# Autodesk Inventor assembly: Chassis-ver10-1111-2019
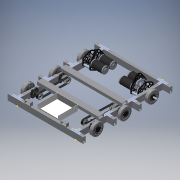
[picture p0: Inventor's stored thumbnail of the model, 180x180]
Saved by Autodesk Inventor 2018 (Build 220112000, 112)
## iProperties
Created: 2019-10-10
Part Number: Chassis-ver10-1111-2019
Document SubType Name: Assembly
Designer: JMHal
Author: JMHal
## Documents named in this file (30)
- F:\GrabCad\2019 - 2020 Off Season\TestChassis\Assembly\Chassis-ver10-1111-2019.iam
- F:\GrabCad\2019 - 2020 Off Season\TestChassis\Parts\2x1 20in Alluminum with Cal Drop.ver1-1111-2019.ipt
- F:\GrabCad\2019 - 2020 Off Season\TestChassis\Parts\2x1 20in Alluminum.ver1-1111-2019.ipt
- F:\GrabCad\2019 - 2020 Off Season\TestChassis\Parts\2x1 2in Alluminum Block.ver1-1111-2019.ipt
- F:\GrabCad\Resources\VEXpro Resources\Bearings\0.5inHexFlangedBearing(1.125inx0.313in)-1111-2016.ipt
- F:\GrabCad\Resources\VEXpro Resources\Versa Motion\VersaBlockKit-1111-2016.ipt
- F:\GrabCad\Resources\VEXpro Resources\Wheels\4 inch\4x1inTractionWheel(Tire)-1111-2016.iam
- F:\GrabCad\Resources\VEXpro Resources\Shafts\0.5inThunderHexShaft(8)-1111-2016.ipt
- F:\GrabCad\Resources\VEXpro Resources\Gearboxes\WCP SS Gearbox\SS-Gearbox.iam
- F:\GrabCad\Resources\VEXpro Resources\Gussets\ChassisGusset-1111-2016.ipt
- F:\GrabCad\2019 - 2020 Off Season\TestChassis\Parts\ElectricalBoardSupport.ver1-1111-2019.ipt
- F:\GrabCad\2019 - 2020 Off Season\TestChassis\Parts\ElectricalBoard.ver1-1111-2019.ipt
- F:\GrabCad\Resources\VEXpro Resources\Spacers\0.5inAcetalSpace(0.5inHex)-1111-2016.ipt
- F:\GrabCad\Resources\VEXpro Resources\Shafts\0.5inThunderHexShaft(8)-1111-2016_MIR.ipt
- F:\GrabCad\Resources\VEXpro Resources\Wheels\4 inch\4x1inTractionWheel(Tire)-1111-2016_MIR.iam
- F:\GrabCad\Resources\VEXpro Resources\Spacers\0.5inAcetalSpace(0.5inHex)-1111-2016_MIR.ipt
- F:\GrabCad\2019 - 2020 Off Season\TestChassis\Parts\BatteryHolder-ver1-1111-2019.ipt
- F:\GrabCad\2019 - 2020 Off Season\TestChassis\Parts\AlluminumSupport-ver1-1111-2019.ipt
- F:\GrabCad\2019 - 2020 Off Season\TestChassis\Parts\Spacer-ver1-1111-2019.ipt
- F:\GrabCad\Resources\VEXpro Resources\Versa Motion\Timing Pulleys\TimingPulley30T15mmDoubleFlange(0.5inHex)-1111-2017.ipt
- F:\GrabCad\Resources\VEXpro Resources\Spacers\0.25inAcetalSpacer(0.5inHex)-1111-2016.ipt
- F:\GrabCad\Resources\VEXpro Resources\Spacers\0.125inAcetalSpacer(0.5inHex)-1111-2016.ipt
- F:\GrabCad\Resources\VEXpro Resources\Spacers\0.0625inAcetalSpacer(0.5inHex)-1111-2016.ipt
- F:\GrabCad\Resources\VEXpro Resources\Spacers\1inAcetalSpacer(0.5inHex)-1111-2016.ipt
- F:\GrabCad\Resources\VEXpro Resources\Versa Motion\Timing Pulleys\TimingPulley30T15mmDoubleFlange(0.5inHex)-1111-2017_MIR.ipt
- F:\GrabCad\Resources\VEXpro Resources\Spacers\0.25inAcetalSpacer(0.5inHex)-1111-2016_MIR.ipt
- F:\GrabCad\Resources\VEXpro Resources\Spacers\0.125inAcetalSpacer(0.5inHex)-1111-2016_MIR.ipt
- F:\GrabCad\Resources\VEXpro Resources\Spacers\0.0625inAcetalSpacer(0.5inHex)-1111-2016_MIR.ipt
- F:\GrabCad\Resources\VEXpro Resources\Spacers\1inAcetalSpacer(0.5inHex)-1111-2016_MIR.ipt
- F:\GrabCad\2019 - 2020 Off Season\TestChassis\Parts\BeltVer1-1111-2019.ipt
## Components (80 placed, 29 different names)
1. 2x1 20in Alluminum with Cal Drop.ver1-1111-2019:1 — Mate:31, Mate:32, Insert:7, Mate:51, Insert:8, Angle:2, Mate:53, Angle:9, Insert:17, Angle:10, Insert:19, Angle:11, Mate:60, Cylindrical:1, Angle:16, Mate:64, Flush:1, Mate:65, Mate:66, Flush:2, Flush:3, Mate:67, Flush:4, Flush:5, Mate:77, Mate:78, Flush:16, Flush:17, Mate:80, Flush:20, Flush:23, Mate:83, Symmetry:1, Flush:43, Mate:101, Mate:102, Symmetry:2
2. 2x1 20in Alluminum.ver1-1111-2019:1 — Mate:65, Mate:66, Flush:2, Flush:3, Mate:68, Mate:72, Mate:81, Flush:22, Mate:82, Flush:24, Mate:98, Flush:44, Mate:105, Mate:106, Flush:54, Flush:55
3. 2x1 20in Alluminum with Cal Drop.ver1-1111-2019:2 — Insert:4, Insert:5, Angle:7, Angle:8, Insert:23, Angle:13, Insert:25, Angle:14, Rotational:1, Angle:17, Flush:6, Mate:70, Flush:8, Mate:73, Mate:74, Flush:9, Mate:85, Flush:30, Flush:31, Flush:32, Flush:34, Flush:35, Flush:36, Flush:37, Symmetry:1, Mate:103, Mate:104, Symmetry:2
4. 0.5inThunderHexShaft(8)-1111-2016:1 — Cylindrical:2, Cylindrical:17, Cylindrical:18, Flush:39
5. SS-Gearbox:1 [sub-assembly] — Rotational:1, Angle:17
6. SS-Gearbox:2 [sub-assembly] — Mate:60, Cylindrical:1, Angle:16, Cylindrical:11, Cylindrical:19, Mate:93
7. 0.5inThunderHexShaft(8)-1111-2016:2 — Cylindrical:3, Cylindrical:15, Cylindrical:16, Flush:38
8. ChassisGusset-1111-2016:1 — Mate:76, Flush:12, Flush:36
9. ChassisGusset-1111-2016:2 — Mate:75, Flush:11, Flush:35
10. ChassisGusset-1111-2016:3 — Mate:78, Flush:14, Flush:17
11. ChassisGusset-1111-2016:4 — Mate:77, Flush:15, Flush:16
12. ChassisGusset-1111-2016:5 — Mate:82, Flush:24, Flush:34
13. ChassisGusset-1111-2016:6 — Mate:81, Flush:22, Flush:23
14. ChassisGusset-1111-2016:7 — Mate:80, Flush:20, Flush:21
15. ChassisGusset-1111-2016:8 — Mate:79, Flush:19, Flush:37
16. ElectricalBoardSupport.ver1-1111-2019:1 — Mate:83, Flush:31, Mate:99, Flush:46, Flush:47, Flush:52, Flush:53
17. ElectricalBoardSupport.ver1-1111-2019:2 — Mate:85, Mate:87, Flush:32, Flush:48, Flush:49, Flush:50, Flush:51
18. ElectricalBoard.ver1-1111-2019:1 — Mate:87, Flush:42, Flush:43, Flush:44, Flush:45
19. 0.5inAcetalSpace(0.5inHex)-1111-2016:1 — Cylindrical:16, Mate:89, Mate:90
20. 0.5inAcetalSpace(0.5inHex)-1111-2016:2 — Cylindrical:18, Mate:91, Mate:92
21. 0.5inAcetalSpace(0.5inHex)-1111-2016:3 — Cylindrical:19, Mate:93, Mate:94
22. 0.5inThunderHexShaft(8)-1111-2016_MIR:1 — Flush:40, Cylindrical:20, Cylindrical:23
23. 0.5inThunderHexShaft(8)-1111-2016_MIR:2 — Flush:41, Cylindrical:21, Cylindrical:22
24. 4x1inTractionWheel(Tire)-1111-2016_MIR:1 [sub-assembly] — Mate:97
25. 4x1inTractionWheel(Tire)-1111-2016_MIR:2 [sub-assembly] — Flush:40, Mate:96, Cylindrical:20
26. 4x1inTractionWheel(Tire)-1111-2016_MIR:3 [sub-assembly] — Flush:41, Mate:95, Cylindrical:21
27. 0.5inAcetalSpace(0.5inHex)-1111-2016_MIR:1 — Mate:95, Cylindrical:22
28. 0.5inAcetalSpace(0.5inHex)-1111-2016_MIR:2 — Mate:96, Cylindrical:23
29. 0.5inAcetalSpace(0.5inHex)-1111-2016_MIR:3 — Mate:97
30. BatteryHolder-ver1-1111-2019:1 — Mate:98, Mate:99, Flush:42, Flush:45
31. AlluminumSupport-ver1-1111-2019:1 — Mate:107, Flush:56, Flush:57
32. AlluminumSupport-ver1-1111-2019:2 — Mate:108, Flush:58, Flush:59
33. Spacer-ver1-1111-2019:1 — Mate:104, Flush:52, Flush:53
34. Spacer-ver1-1111-2019:2 — Mate:103, Flush:50, Flush:51
35. Spacer-ver1-1111-2019:3 — Mate:101, Flush:46, Flush:47
36. Spacer-ver1-1111-2019:4 — Mate:102, Flush:48, Flush:49
37. Spacer-ver1-1111-2019:5 — Mate:105, Flush:55, Mate:107, Flush:56, Flush:57
38. Spacer-ver1-1111-2019:6 — Mate:106, Flush:54, Mate:108, Flush:58, Flush:59
39. TimingPulley30T15mmDoubleFlange(0.5inHex)-1111-2017:1 — Rotational:7, Mate:117
40. TimingPulley30T15mmDoubleFlange(0.5inHex)-1111-2017:2 — Rotational:3, Mate:118
41. TimingPulley30T15mmDoubleFlange(0.5inHex)-1111-2017:3 — Cylindrical:25, Mate:111, Rotational:2
42. 0.25inAcetalSpacer(0.5inHex)-1111-2016:1 — Cylindrical:25, Cylindrical:26, Mate:109, Mate:110, Rotational:4
43. 0.125inAcetalSpacer(0.5inHex)-1111-2016:1 — Cylindrical:26, Mate:110, Mate:111
44. 0.0625inAcetalSpacer(0.5inHex)-1111-2016:1 — Rotational:2, Rotational:3
45. 0.25inAcetalSpacer(0.5inHex)-1111-2016:2 — Rotational:6, Rotational:7
46. 1inAcetalSpacer(0.5inHex)-1111-2016:1 — Rotational:5, Rotational:6
47. TimingPulley30T15mmDoubleFlange(0.5inHex)-1111-2017_MIR:1 — Rotational:10, Mate:114, Mate:115
48. TimingPulley30T15mmDoubleFlange(0.5inHex)-1111-2017_MIR:2 — Rotational:8, Mate:116
49. TimingPulley30T15mmDoubleFlange(0.5inHex)-1111-2017_MIR:3 — Mate:112, Cylindrical:27, Rotational:9
50. 0.25inAcetalSpacer(0.5inHex)-1111-2016_MIR:1 — Mate:113, Cylindrical:27, Cylindrical:28, Rotational:12
51. 0.125inAcetalSpacer(0.5inHex)-1111-2016_MIR:1 — Mate:112, Mate:113, Cylindrical:28
52. 0.0625inAcetalSpacer(0.5inHex)-1111-2016_MIR:1 — Rotational:8, Rotational:9
53. 0.25inAcetalSpacer(0.5inHex)-1111-2016_MIR:2 — Rotational:10, Rotational:11
54. 1inAcetalSpacer(0.5inHex)-1111-2016_MIR:1 — Rotational:11, Rotational:13
55. BeltVer1-1111-2019:1 — Mate:114, Mate:115, Mate:116
56. BeltVer1-1111-2019:2 — Mate:117, Mate:118
57. 0.5inHexFlangedBearing(1.125inx0.313in)-1111-2016:20 — Rotational:12
58. 0.5inHexFlangedBearing(1.125inx0.313in)-1111-2016:19 — Rotational:13
59. 0.5inHexFlangedBearing(1.125inx0.313in)-1111-2016:6 — Insert:4, Mate:46, Mate:47
60. 0.5inHexFlangedBearing(1.125inx0.313in)-1111-2016:7 — Insert:5, Mate:48, Mate:49
61. 0.5inHexFlangedBearing(1.125inx0.313in)-1111-2016:17 — Insert:19, Cylindrical:3, Rotational:5
62. 0.5inHexFlangedBearing(1.125inx0.313in)-1111-2016:16 — Insert:16, Insert:17, Cylindrical:2, Mate:109, Rotational:4
63. 0.5inHexFlangedBearing(1.125inx0.313in)-1111-2016:9 — Insert:7, Mate:50, Mate:91
64. 0.5inHexFlangedBearing(1.125inx0.313in)-1111-2016:10 — Insert:8, Mate:52, Mate:89
65. 2x1 2in Alluminum Block.ver1-1111-2019:5 — Mate:31, Mate:32, Mate:69, Flush:15
66. 2x1 2in Alluminum Block.ver1-1111-2019:6 — Mate:64, Flush:1, Mate:68, Flush:14
67. 2x1 2in Alluminum Block.ver1-1111-2019:7 — Mate:72, Mate:74, Flush:9, Mate:75, Flush:11
68. 2x1 2in Alluminum Block.ver1-1111-2019:8 — Mate:70, Flush:8, Mate:71, Mate:76, Flush:12
69. VersaBlockKit-1111-2016:2 — Mate:46, Mate:47, Angle:8
70. VersaBlockKit-1111-2016:3 — Mate:48, Mate:49, Angle:7
71. VersaBlockKit-1111-2016:5 — Mate:50, Mate:51, Angle:2
72. VersaBlockKit-1111-2016:6 — Mate:52, Mate:53, Angle:9
73. VersaBlockKit-1111-2016:8 — Insert:16, Angle:10
74. VersaBlockKit-1111-2016:9 — Angle:11
75. VersaBlockKit-1111-2016:11 — Insert:23, Angle:13
76. VersaBlockKit-1111-2016:12 — Insert:25, Angle:14
77. 2x1 20in Alluminum.ver1-1111-2019:2 — Mate:67, Flush:4, Flush:5, Mate:69, Flush:6, Mate:71, Mate:73, Mate:79, Flush:19, Flush:21, Flush:30
78. 4x1inTractionWheel(Tire)-1111-2016:4 [sub-assembly] — Cylindrical:11, Mate:94
79. 4x1inTractionWheel(Tire)-1111-2016:5 [sub-assembly] — Cylindrical:17, Mate:92, Flush:39
80. 4x1inTractionWheel(Tire)-1111-2016:6 [sub-assembly] — Cylindrical:15, Mate:90, Flush:38
## Relationships (169: Mate 66, Flush 49, CylindricalJoint 17, RevoluteJoint 13, Insert 12, Angle 10, Symmetry 2)
- Mate:31: 2x1 20in Alluminum with Cal Drop.ver1-1111-2019:1 ↔ 2x1 2in Alluminum Block.ver1-1111-2019:5
- Mate:32: 2x1 20in Alluminum with Cal Drop.ver1-1111-2019:1 ↔ 2x1 2in Alluminum Block.ver1-1111-2019:5
- Insert:4: 2x1 20in Alluminum with Cal Drop.ver1-1111-2019:2 ↔ 0.5inHexFlangedBearing(1.125inx0.313in)-1111-2016:6
- Mate:46: 0.5inHexFlangedBearing(1.125inx0.313in)-1111-2016:6 ↔ VersaBlockKit-1111-2016:2
- Mate:47: 0.5inHexFlangedBearing(1.125inx0.313in)-1111-2016:6 ↔ VersaBlockKit-1111-2016:2
- Insert:5: 2x1 20in Alluminum with Cal Drop.ver1-1111-2019:2 ↔ 0.5inHexFlangedBearing(1.125inx0.313in)-1111-2016:7
- Mate:48: 0.5inHexFlangedBearing(1.125inx0.313in)-1111-2016:7 ↔ VersaBlockKit-1111-2016:3
- Mate:49: 0.5inHexFlangedBearing(1.125inx0.313in)-1111-2016:7 ↔ VersaBlockKit-1111-2016:3
- Insert:7: 2x1 20in Alluminum with Cal Drop.ver1-1111-2019:1 ↔ 0.5inHexFlangedBearing(1.125inx0.313in)-1111-2016:9
- Mate:50: 0.5inHexFlangedBearing(1.125inx0.313in)-1111-2016:9 ↔ VersaBlockKit-1111-2016:5
- Mate:51: 2x1 20in Alluminum with Cal Drop.ver1-1111-2019:1 ↔ VersaBlockKit-1111-2016:5
- Insert:8: 2x1 20in Alluminum with Cal Drop.ver1-1111-2019:1 ↔ 0.5inHexFlangedBearing(1.125inx0.313in)-1111-2016:10
- Angle:2 (0 deg): 2x1 20in Alluminum with Cal Drop.ver1-1111-2019:1 ↔ VersaBlockKit-1111-2016:5
- Angle:7 (0 deg): 2x1 20in Alluminum with Cal Drop.ver1-1111-2019:2 ↔ VersaBlockKit-1111-2016:3
- Angle:8 (0 deg): 2x1 20in Alluminum with Cal Drop.ver1-1111-2019:2 ↔ VersaBlockKit-1111-2016:2
- Mate:52: 0.5inHexFlangedBearing(1.125inx0.313in)-1111-2016:10 ↔ VersaBlockKit-1111-2016:6
- Mate:53: 2x1 20in Alluminum with Cal Drop.ver1-1111-2019:1 ↔ VersaBlockKit-1111-2016:6
- Angle:9 (0 deg): 2x1 20in Alluminum with Cal Drop.ver1-1111-2019:1 ↔ VersaBlockKit-1111-2016:6
- [Mate]: 0.5inHexFlangedBearing(1.125inx0.313in)-1111-2016:16 ↔ VersaBlockKit-1111-2016:8
- Insert:16: 0.5inHexFlangedBearing(1.125inx0.313in)-1111-2016:16 ↔ VersaBlockKit-1111-2016:8
- Insert:17: 2x1 20in Alluminum with Cal Drop.ver1-1111-2019:1 ↔ 0.5inHexFlangedBearing(1.125inx0.313in)-1111-2016:16
- Angle:10 (0 deg): 2x1 20in Alluminum with Cal Drop.ver1-1111-2019:1 ↔ VersaBlockKit-1111-2016:8
- [Mate]: 0.5inHexFlangedBearing(1.125inx0.313in)-1111-2016:17 ↔ VersaBlockKit-1111-2016:9
- [Insert]: 0.5inHexFlangedBearing(1.125inx0.313in)-1111-2016:17 ↔ VersaBlockKit-1111-2016:9
- Insert:19: 2x1 20in Alluminum with Cal Drop.ver1-1111-2019:1 ↔ 0.5inHexFlangedBearing(1.125inx0.313in)-1111-2016:17
- Angle:11 (0 deg): 2x1 20in Alluminum with Cal Drop.ver1-1111-2019:1 ↔ VersaBlockKit-1111-2016:9
- [Mate]: 0.5inHexFlangedBearing(1.125inx0.313in)-1111-2016:19 ↔ VersaBlockKit-1111-2016:11
- [Insert]: 0.5inHexFlangedBearing(1.125inx0.313in)-1111-2016:19 ↔ VersaBlockKit-1111-2016:11
- Insert:23: 2x1 20in Alluminum with Cal Drop.ver1-1111-2019:2 ↔ VersaBlockKit-1111-2016:11
- Angle:13 (0 deg): 2x1 20in Alluminum with Cal Drop.ver1-1111-2019:2 ↔ VersaBlockKit-1111-2016:11
- [Mate]: 0.5inHexFlangedBearing(1.125inx0.313in)-1111-2016:20 ↔ VersaBlockKit-1111-2016:12
- [Insert]: 0.5inHexFlangedBearing(1.125inx0.313in)-1111-2016:20 ↔ VersaBlockKit-1111-2016:12
- Insert:25: 2x1 20in Alluminum with Cal Drop.ver1-1111-2019:2 ↔ VersaBlockKit-1111-2016:12
- Angle:14 (0 deg): 2x1 20in Alluminum with Cal Drop.ver1-1111-2019:2 ↔ VersaBlockKit-1111-2016:12
- Mate:60: 2x1 20in Alluminum with Cal Drop.ver1-1111-2019:1 ↔ SS-Gearbox:2
- Cylindrical:1: 2x1 20in Alluminum with Cal Drop.ver1-1111-2019:1 ↔ SS-Gearbox:2
- Cylindrical:2: 0.5inThunderHexShaft(8)-1111-2016:1 ↔ 0.5inHexFlangedBearing(1.125inx0.313in)-1111-2016:16
- Cylindrical:3: 0.5inThunderHexShaft(8)-1111-2016:2 ↔ 0.5inHexFlangedBearing(1.125inx0.313in)-1111-2016:17
- Angle:16 (90 deg): 2x1 20in Alluminum with Cal Drop.ver1-1111-2019:1 ↔ SS-Gearbox:2
- Rotational:1 [RevoluteJoint]: 2x1 20in Alluminum with Cal Drop.ver1-1111-2019:2 ↔ SS-Gearbox:1
- Angle:17 (90 deg): 2x1 20in Alluminum with Cal Drop.ver1-1111-2019:2 ↔ SS-Gearbox:1
- Cylindrical:11: SS-Gearbox:2 ↔ 4x1inTractionWheel(Tire)-1111-2016:4
- Cylindrical:17: 0.5inThunderHexShaft(8)-1111-2016:1 ↔ 4x1inTractionWheel(Tire)-1111-2016:5
- Cylindrical:15: 0.5inThunderHexShaft(8)-1111-2016:2 ↔ 4x1inTractionWheel(Tire)-1111-2016:6
- Mate:64: 2x1 20in Alluminum with Cal Drop.ver1-1111-2019:1 ↔ 2x1 2in Alluminum Block.ver1-1111-2019:6
- Flush:1: 2x1 20in Alluminum with Cal Drop.ver1-1111-2019:1 ↔ 2x1 2in Alluminum Block.ver1-1111-2019:6
- Mate:65: 2x1 20in Alluminum with Cal Drop.ver1-1111-2019:1 ↔ 2x1 20in Alluminum.ver1-1111-2019:1
- Mate:66: 2x1 20in Alluminum with Cal Drop.ver1-1111-2019:1 ↔ 2x1 20in Alluminum.ver1-1111-2019:1
- Flush:2: 2x1 20in Alluminum with Cal Drop.ver1-1111-2019:1 ↔ 2x1 20in Alluminum.ver1-1111-2019:1
- Flush:3 (63.5 mm): 2x1 20in Alluminum with Cal Drop.ver1-1111-2019:1 ↔ 2x1 20in Alluminum.ver1-1111-2019:1
- Mate:67: 2x1 20in Alluminum with Cal Drop.ver1-1111-2019:1 ↔ 2x1 20in Alluminum.ver1-1111-2019:2
- Flush:4: 2x1 20in Alluminum with Cal Drop.ver1-1111-2019:1 ↔ 2x1 20in Alluminum.ver1-1111-2019:2
- Flush:5 (-63.5 mm): 2x1 20in Alluminum with Cal Drop.ver1-1111-2019:1 ↔ 2x1 20in Alluminum.ver1-1111-2019:2
- Mate:68 (254 mm): 2x1 20in Alluminum.ver1-1111-2019:1 ↔ 2x1 2in Alluminum Block.ver1-1111-2019:6
- Mate:69 (254 mm): 2x1 2in Alluminum Block.ver1-1111-2019:5 ↔ 2x1 20in Alluminum.ver1-1111-2019:2
- Flush:6: 2x1 20in Alluminum with Cal Drop.ver1-1111-2019:2 ↔ 2x1 20in Alluminum.ver1-1111-2019:2
- Mate:70: 2x1 20in Alluminum with Cal Drop.ver1-1111-2019:2 ↔ 2x1 2in Alluminum Block.ver1-1111-2019:8
- Flush:8: 2x1 20in Alluminum with Cal Drop.ver1-1111-2019:2 ↔ 2x1 2in Alluminum Block.ver1-1111-2019:8
- Mate:71 (254 mm): 2x1 2in Alluminum Block.ver1-1111-2019:8 ↔ 2x1 20in Alluminum.ver1-1111-2019:2
- Mate:72 (254 mm): 2x1 20in Alluminum.ver1-1111-2019:1 ↔ 2x1 2in Alluminum Block.ver1-1111-2019:7
- Mate:73: 2x1 20in Alluminum with Cal Drop.ver1-1111-2019:2 ↔ 2x1 20in Alluminum.ver1-1111-2019:2
- Mate:74: 2x1 20in Alluminum with Cal Drop.ver1-1111-2019:2 ↔ 2x1 2in Alluminum Block.ver1-1111-2019:7
- Flush:9: 2x1 20in Alluminum with Cal Drop.ver1-1111-2019:2 ↔ 2x1 2in Alluminum Block.ver1-1111-2019:7
- Mate:75: ChassisGusset-1111-2016:2 ↔ 2x1 2in Alluminum Block.ver1-1111-2019:7
- Flush:11: ChassisGusset-1111-2016:2 ↔ 2x1 2in Alluminum Block.ver1-1111-2019:7
- Mate:76: ChassisGusset-1111-2016:1 ↔ 2x1 2in Alluminum Block.ver1-1111-2019:8
- Flush:12: ChassisGusset-1111-2016:1 ↔ 2x1 2in Alluminum Block.ver1-1111-2019:8
- Mate:77: 2x1 20in Alluminum with Cal Drop.ver1-1111-2019:1 ↔ ChassisGusset-1111-2016:4
- Mate:78: 2x1 20in Alluminum with Cal Drop.ver1-1111-2019:1 ↔ ChassisGusset-1111-2016:3
- Flush:14: ChassisGusset-1111-2016:3 ↔ 2x1 2in Alluminum Block.ver1-1111-2019:6
- Flush:15: ChassisGusset-1111-2016:4 ↔ 2x1 2in Alluminum Block.ver1-1111-2019:5
- Flush:16: 2x1 20in Alluminum with Cal Drop.ver1-1111-2019:1 ↔ ChassisGusset-1111-2016:4
- Flush:17: 2x1 20in Alluminum with Cal Drop.ver1-1111-2019:1 ↔ ChassisGusset-1111-2016:3
- Mate:79: ChassisGusset-1111-2016:8 ↔ 2x1 20in Alluminum.ver1-1111-2019:2
- Flush:19: ChassisGusset-1111-2016:8 ↔ 2x1 20in Alluminum.ver1-1111-2019:2
- Mate:80: 2x1 20in Alluminum with Cal Drop.ver1-1111-2019:1 ↔ ChassisGusset-1111-2016:7
- Flush:20: 2x1 20in Alluminum with Cal Drop.ver1-1111-2019:1 ↔ ChassisGusset-1111-2016:7
- Flush:21: ChassisGusset-1111-2016:7 ↔ 2x1 20in Alluminum.ver1-1111-2019:2
- Mate:81: 2x1 20in Alluminum.ver1-1111-2019:1 ↔ ChassisGusset-1111-2016:6
- Flush:22: 2x1 20in Alluminum.ver1-1111-2019:1 ↔ ChassisGusset-1111-2016:6
- Flush:23: 2x1 20in Alluminum with Cal Drop.ver1-1111-2019:1 ↔ ChassisGusset-1111-2016:6
- Mate:82: 2x1 20in Alluminum.ver1-1111-2019:1 ↔ ChassisGusset-1111-2016:5
- Flush:24: 2x1 20in Alluminum.ver1-1111-2019:1 ↔ ChassisGusset-1111-2016:5
- Mate:83 (3.175 mm): 2x1 20in Alluminum with Cal Drop.ver1-1111-2019:1 ↔ ElectricalBoardSupport.ver1-1111-2019:1
- Mate:85 (3.175 mm): 2x1 20in Alluminum with Cal Drop.ver1-1111-2019:2 ↔ ElectricalBoardSupport.ver1-1111-2019:2
- Mate:87: ElectricalBoardSupport.ver1-1111-2019:2 ↔ ElectricalBoard.ver1-1111-2019:1
- Flush:30 (63.5 mm): 2x1 20in Alluminum with Cal Drop.ver1-1111-2019:2 ↔ 2x1 20in Alluminum.ver1-1111-2019:2
- Flush:31: 2x1 20in Alluminum with Cal Drop.ver1-1111-2019:2 ↔ ElectricalBoardSupport.ver1-1111-2019:1
- Flush:32: 2x1 20in Alluminum with Cal Drop.ver1-1111-2019:2 ↔ ElectricalBoardSupport.ver1-1111-2019:2
- Flush:34: 2x1 20in Alluminum with Cal Drop.ver1-1111-2019:2 ↔ ChassisGusset-1111-2016:5
- Flush:35: 2x1 20in Alluminum with Cal Drop.ver1-1111-2019:2 ↔ ChassisGusset-1111-2016:2
- Flush:36: 2x1 20in Alluminum with Cal Drop.ver1-1111-2019:2 ↔ ChassisGusset-1111-2016:1
- Flush:37: 2x1 20in Alluminum with Cal Drop.ver1-1111-2019:2 ↔ ChassisGusset-1111-2016:8
- Cylindrical:16: 0.5inThunderHexShaft(8)-1111-2016:2 ↔ 0.5inAcetalSpace(0.5inHex)-1111-2016:1
- Mate:89: 0.5inAcetalSpace(0.5inHex)-1111-2016:1 ↔ 0.5inHexFlangedBearing(1.125inx0.313in)-1111-2016:10
- Mate:90: 0.5inAcetalSpace(0.5inHex)-1111-2016:1 ↔ 4x1inTractionWheel(Tire)-1111-2016:6
- Flush:38: 0.5inThunderHexShaft(8)-1111-2016:2 ↔ 4x1inTractionWheel(Tire)-1111-2016:6
- Cylindrical:18: 0.5inThunderHexShaft(8)-1111-2016:1 ↔ 0.5inAcetalSpace(0.5inHex)-1111-2016:2
- Mate:91: 0.5inAcetalSpace(0.5inHex)-1111-2016:2 ↔ 0.5inHexFlangedBearing(1.125inx0.313in)-1111-2016:9
- Mate:92: 0.5inAcetalSpace(0.5inHex)-1111-2016:2 ↔ 4x1inTractionWheel(Tire)-1111-2016:5
- Flush:39: 0.5inThunderHexShaft(8)-1111-2016:1 ↔ 4x1inTractionWheel(Tire)-1111-2016:5
- Cylindrical:19: SS-Gearbox:2 ↔ 0.5inAcetalSpace(0.5inHex)-1111-2016:3
- Mate:93: SS-Gearbox:2 ↔ 0.5inAcetalSpace(0.5inHex)-1111-2016:3
- Mate:94: 0.5inAcetalSpace(0.5inHex)-1111-2016:3 ↔ 4x1inTractionWheel(Tire)-1111-2016:4
- Symmetry:1: 2x1 20in Alluminum with Cal Drop.ver1-1111-2019:1 ↔ 2x1 20in Alluminum with Cal Drop.ver1-1111-2019:2
- Flush:40: 0.5inThunderHexShaft(8)-1111-2016_MIR:1 ↔ 4x1inTractionWheel(Tire)-1111-2016_MIR:2
- Flush:41: 0.5inThunderHexShaft(8)-1111-2016_MIR:2 ↔ 4x1inTractionWheel(Tire)-1111-2016_MIR:3
- Mate:95: 4x1inTractionWheel(Tire)-1111-2016_MIR:3 ↔ 0.5inAcetalSpace(0.5inHex)-1111-2016_MIR:1
- Mate:96: 4x1inTractionWheel(Tire)-1111-2016_MIR:2 ↔ 0.5inAcetalSpace(0.5inHex)-1111-2016_MIR:2
- Mate:97: 4x1inTractionWheel(Tire)-1111-2016_MIR:1 ↔ 0.5inAcetalSpace(0.5inHex)-1111-2016_MIR:3
- Cylindrical:20: 0.5inThunderHexShaft(8)-1111-2016_MIR:1 ↔ 4x1inTractionWheel(Tire)-1111-2016_MIR:2
- Cylindrical:21: 0.5inThunderHexShaft(8)-1111-2016_MIR:2 ↔ 4x1inTractionWheel(Tire)-1111-2016_MIR:3
- Cylindrical:22: 0.5inThunderHexShaft(8)-1111-2016_MIR:2 ↔ 0.5inAcetalSpace(0.5inHex)-1111-2016_MIR:1
- Cylindrical:23: 0.5inThunderHexShaft(8)-1111-2016_MIR:1 ↔ 0.5inAcetalSpace(0.5inHex)-1111-2016_MIR:2
- Mate:98: 2x1 20in Alluminum.ver1-1111-2019:1 ↔ BatteryHolder-ver1-1111-2019:1
- Mate:99: ElectricalBoardSupport.ver1-1111-2019:1 ↔ BatteryHolder-ver1-1111-2019:1
- Flush:42: ElectricalBoard.ver1-1111-2019:1 ↔ BatteryHolder-ver1-1111-2019:1
- Flush:43: 2x1 20in Alluminum with Cal Drop.ver1-1111-2019:1 ↔ ElectricalBoard.ver1-1111-2019:1
- Flush:44: 2x1 20in Alluminum.ver1-1111-2019:1 ↔ ElectricalBoard.ver1-1111-2019:1
- Flush:45: ElectricalBoard.ver1-1111-2019:1 ↔ BatteryHolder-ver1-1111-2019:1
- Mate:101: 2x1 20in Alluminum with Cal Drop.ver1-1111-2019:1 ↔ Spacer-ver1-1111-2019:3
- Flush:46: ElectricalBoardSupport.ver1-1111-2019:1 ↔ Spacer-ver1-1111-2019:3
- Flush:47: ElectricalBoardSupport.ver1-1111-2019:1 ↔ Spacer-ver1-1111-2019:3
- Mate:102: 2x1 20in Alluminum with Cal Drop.ver1-1111-2019:1 ↔ Spacer-ver1-1111-2019:4
- Flush:48: ElectricalBoardSupport.ver1-1111-2019:2 ↔ Spacer-ver1-1111-2019:4
- Flush:49: ElectricalBoardSupport.ver1-1111-2019:2 ↔ Spacer-ver1-1111-2019:4
- Mate:103: 2x1 20in Alluminum with Cal Drop.ver1-1111-2019:2 ↔ Spacer-ver1-1111-2019:2
- Flush:50: ElectricalBoardSupport.ver1-1111-2019:2 ↔ Spacer-ver1-1111-2019:2
- Flush:51: ElectricalBoardSupport.ver1-1111-2019:2 ↔ Spacer-ver1-1111-2019:2
- Mate:104: 2x1 20in Alluminum with Cal Drop.ver1-1111-2019:2 ↔ Spacer-ver1-1111-2019:1
- Flush:52: ElectricalBoardSupport.ver1-1111-2019:1 ↔ Spacer-ver1-1111-2019:1
- Flush:53: ElectricalBoardSupport.ver1-1111-2019:1 ↔ Spacer-ver1-1111-2019:1
- Mate:105: 2x1 20in Alluminum.ver1-1111-2019:1 ↔ Spacer-ver1-1111-2019:5
- Mate:106: 2x1 20in Alluminum.ver1-1111-2019:1 ↔ Spacer-ver1-1111-2019:6
- Flush:54: 2x1 20in Alluminum.ver1-1111-2019:1 ↔ Spacer-ver1-1111-2019:6
- Flush:55: 2x1 20in Alluminum.ver1-1111-2019:1 ↔ Spacer-ver1-1111-2019:5
- Mate:107: AlluminumSupport-ver1-1111-2019:1 ↔ Spacer-ver1-1111-2019:5
- Flush:56: AlluminumSupport-ver1-1111-2019:1 ↔ Spacer-ver1-1111-2019:5
- Flush:57: AlluminumSupport-ver1-1111-2019:1 ↔ Spacer-ver1-1111-2019:5
- Mate:108: AlluminumSupport-ver1-1111-2019:2 ↔ Spacer-ver1-1111-2019:6
- Flush:58: AlluminumSupport-ver1-1111-2019:2 ↔ Spacer-ver1-1111-2019:6
- Flush:59: AlluminumSupport-ver1-1111-2019:2 ↔ Spacer-ver1-1111-2019:6
- Cylindrical:25: TimingPulley30T15mmDoubleFlange(0.5inHex)-1111-2017:3 ↔ 0.25inAcetalSpacer(0.5inHex)-1111-2016:1
- Cylindrical:26: 0.25inAcetalSpacer(0.5inHex)-1111-2016:1 ↔ 0.125inAcetalSpacer(0.5inHex)-1111-2016:1
- Mate:109: 0.25inAcetalSpacer(0.5inHex)-1111-2016:1 ↔ 0.5inHexFlangedBearing(1.125inx0.313in)-1111-2016:16
- Mate:110: 0.25inAcetalSpacer(0.5inHex)-1111-2016:1 ↔ 0.125inAcetalSpacer(0.5inHex)-1111-2016:1
- Mate:111: TimingPulley30T15mmDoubleFlange(0.5inHex)-1111-2017:3 ↔ 0.125inAcetalSpacer(0.5inHex)-1111-2016:1
- Rotational:2 [RevoluteJoint]: TimingPulley30T15mmDoubleFlange(0.5inHex)-1111-2017:3 ↔ 0.0625inAcetalSpacer(0.5inHex)-1111-2016:1
- Rotational:3 [RevoluteJoint]: TimingPulley30T15mmDoubleFlange(0.5inHex)-1111-2017:2 ↔ 0.0625inAcetalSpacer(0.5inHex)-1111-2016:1
- Rotational:4 [RevoluteJoint]: 0.25inAcetalSpacer(0.5inHex)-1111-2016:1 ↔ 0.5inHexFlangedBearing(1.125inx0.313in)-1111-2016:16
- Rotational:5 [RevoluteJoint]: 1inAcetalSpacer(0.5inHex)-1111-2016:1 ↔ 0.5inHexFlangedBearing(1.125inx0.313in)-1111-2016:17
- Rotational:6 [RevoluteJoint]: 0.25inAcetalSpacer(0.5inHex)-1111-2016:2 ↔ 1inAcetalSpacer(0.5inHex)-1111-2016:1
- Rotational:7 [RevoluteJoint]: TimingPulley30T15mmDoubleFlange(0.5inHex)-1111-2017:1 ↔ 0.25inAcetalSpacer(0.5inHex)-1111-2016:2
- Symmetry:2: 2x1 20in Alluminum with Cal Drop.ver1-1111-2019:1 ↔ 2x1 20in Alluminum with Cal Drop.ver1-1111-2019:2
- Mate:112: TimingPulley30T15mmDoubleFlange(0.5inHex)-1111-2017_MIR:3 ↔ 0.125inAcetalSpacer(0.5inHex)-1111-2016_MIR:1
- Mate:113: 0.25inAcetalSpacer(0.5inHex)-1111-2016_MIR:1 ↔ 0.125inAcetalSpacer(0.5inHex)-1111-2016_MIR:1
- Cylindrical:27: TimingPulley30T15mmDoubleFlange(0.5inHex)-1111-2017_MIR:3 ↔ 0.25inAcetalSpacer(0.5inHex)-1111-2016_MIR:1
- Cylindrical:28: 0.25inAcetalSpacer(0.5inHex)-1111-2016_MIR:1 ↔ 0.125inAcetalSpacer(0.5inHex)-1111-2016_MIR:1
- Rotational:8 [RevoluteJoint]: TimingPulley30T15mmDoubleFlange(0.5inHex)-1111-2017_MIR:2 ↔ 0.0625inAcetalSpacer(0.5inHex)-1111-2016_MIR:1
- Rotational:9 [RevoluteJoint]: TimingPulley30T15mmDoubleFlange(0.5inHex)-1111-2017_MIR:3 ↔ 0.0625inAcetalSpacer(0.5inHex)-1111-2016_MIR:1
- Rotational:10 [RevoluteJoint]: TimingPulley30T15mmDoubleFlange(0.5inHex)-1111-2017_MIR:1 ↔ 0.25inAcetalSpacer(0.5inHex)-1111-2016_MIR:2
- Rotational:11 [RevoluteJoint]: 0.25inAcetalSpacer(0.5inHex)-1111-2016_MIR:2 ↔ 1inAcetalSpacer(0.5inHex)-1111-2016_MIR:1
- Rotational:12 [RevoluteJoint]: 0.25inAcetalSpacer(0.5inHex)-1111-2016_MIR:1 ↔ 0.5inHexFlangedBearing(1.125inx0.313in)-1111-2016:20
- Rotational:13 [RevoluteJoint]: 1inAcetalSpacer(0.5inHex)-1111-2016_MIR:1 ↔ 0.5inHexFlangedBearing(1.125inx0.313in)-1111-2016:19
- Mate:114: TimingPulley30T15mmDoubleFlange(0.5inHex)-1111-2017_MIR:1 ↔ BeltVer1-1111-2019:1
- Mate:115: TimingPulley30T15mmDoubleFlange(0.5inHex)-1111-2017_MIR:1 ↔ BeltVer1-1111-2019:1
- Mate:116: TimingPulley30T15mmDoubleFlange(0.5inHex)-1111-2017_MIR:2 ↔ BeltVer1-1111-2019:1
- Mate:117: TimingPulley30T15mmDoubleFlange(0.5inHex)-1111-2017:1 ↔ BeltVer1-1111-2019:2
- Mate:118: TimingPulley30T15mmDoubleFlange(0.5inHex)-1111-2017:2 ↔ BeltVer1-1111-2019:2
## Named parameters: d89_d76 = 0 mm, d93_d89_d76 = 0 mm, d94_d90 = 0 mm, d103_d89_d76 = 0 mm, d104_d90 = 0 mm, d107_d89_d76 = 0 mm, d108_d90 = 0 mm
